# Autodesk Inventor assembly: Syringe
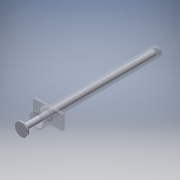
[picture p0: Inventor's stored thumbnail of the model, 180x180]
Saved by Autodesk Inventor 2016 (Build 200138000, 138)
## iProperties
Created: 2017-02-18
Part Number: Syringe
Document SubType Name: Assembly
Designer: Owner
Author: Owner
## Documents named in this file (3)
- C:\Users\Owner\Documents\Inventor\TSA\2017\Animatronics\Alligator\Syringe1mL\Syringe.iam
- C:\Users\Owner\Documents\Inventor\TSA\2017\Animatronics\Alligator\Syringe1mL\SyringEnd.ipt
- C:\Users\Owner\Documents\Inventor\TSA\2017\Animatronics\Alligator\Syringe1mL\SyringeBody.ipt
## Components (2 placed, 2 different names)
1. SyringEnd:1 — Mate:1
2. SyringeBody:1 — Mate:1
## Relationships (1: Mate 1)
- Mate:1: SyringEnd:1 ↔ SyringeBody:1
